# Autodesk Inventor assembly: prototype3
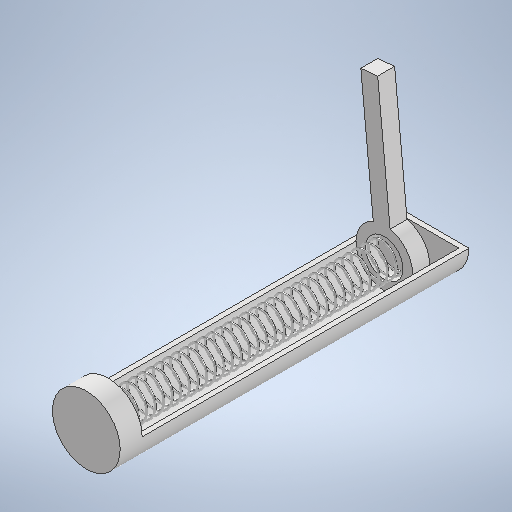
[picture p0: Inventor's stored thumbnail of the model, 512x512]
Saved by Autodesk Inventor 2025.1 (Build 291241020, 241B)
## iProperties
Created: 2024-11-22
Part Number: prototype3
Document SubType Name: Assembly
Designer: leon-
Author: leon-
## Documents named in this file (4)
- C:\Users\leon-\OneDrive\Dokumente\Education\Berkeley\Embedded_Systems\Project\MagDrop4\CAD_Model\3DPrint_Parts\Magazine_Test\prototype3.iam
- C:\Users\leon-\OneDrive\Dokumente\Education\Berkeley\Embedded_Systems\Project\MagDrop4\CAD_Model\3DPrint_Parts\Magazine_Test\prototype3_1.ipt
- C:\Users\leon-\OneDrive\Dokumente\Education\Berkeley\Embedded_Systems\Project\MagDrop4\CAD_Model\Purchase_Parts\Mechanical\Spring.ipt
- C:\Users\leon-\OneDrive\Dokumente\Education\Berkeley\Embedded_Systems\Project\MagDrop4\CAD_Model\3DPrint_Parts\Magazine_Test\prototype3_2.ipt
## Components (3 placed, 3 different names)
1. prototype3_1:1 — Mate:1, Mate:2, Mate:3
2. Spring:1 — Mate:1, Mate:2, Mate:4
3. prototype3_2:1 — Mate:3, Mate:4
## Relationships (4: Mate 4)
- Mate:1: prototype3_1:1 ↔ Spring:1
- Mate:2: prototype3_1:1 ↔ Spring:1
- Mate:3: prototype3_1:1 ↔ prototype3_2:1
- Mate:4: Spring:1 ↔ prototype3_2:1
